# Autodesk Inventor assembly: __VK_Stopper_Vor-Stopper_Einheit_erweitert
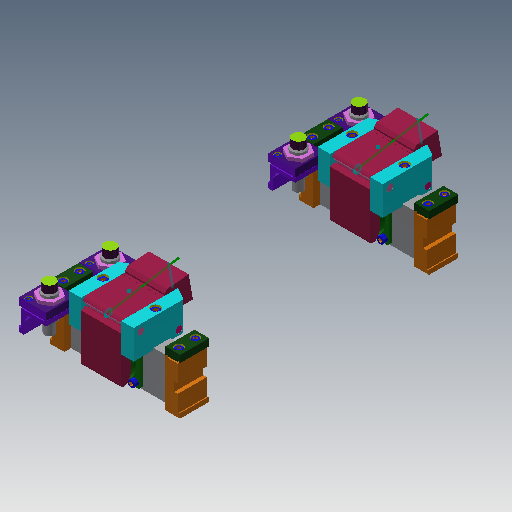
[picture p0: Inventor's stored thumbnail of the model, 512x512]
Saved by Autodesk Inventor 2025.1 (Build 291241000, 241)
## iProperties
Created: 2023-11-18
Part Number: __VK_Stopper_Vor-Stopper_Einheit_erweitert
Material: Generisch
Document SubType Name: Assembly
Designer: RP
Author: RP
## Documents named in this file (2)
- C:\Users\Erik\Erik\Hochschule\3. Semester\CAD\CAD-Paspa\Useless Box\_Verkettung\__VK_Stopper_Vor-Stopper_Einheit_erweitert.iam
- C:\Users\Erik\Erik\Hochschule\3. Semester\CAD\CAD-Paspa\Useless Box\_Verkettung\__VK_Stopper_Einheit.iam
## Components (2 placed, 1 different names)
1. __VK_Stopper_Einheit:1 [sub-assembly] — Fluchtend:1, Fluchtend:2, Fluchtend:3, Fluchtend:6
2. __VK_Stopper_Einheit:2 [sub-assembly] — Fluchtend:4, Fluchtend:5, Fluchtend:6
## Relationships (6: Flush 6)
- Fluchtend:1 [Flush]: __VK_Stopper_Einheit:1
- Fluchtend:2 [Flush]: __VK_Stopper_Einheit:1
- Fluchtend:3 [Flush]: __VK_Stopper_Einheit:1
- Fluchtend:4 [Flush]: __VK_Stopper_Einheit:2
- Fluchtend:5 [Flush]: __VK_Stopper_Einheit:2
- Fluchtend:6 [Flush] (300 mm): __VK_Stopper_Einheit:1 ↔ __VK_Stopper_Einheit:2
